# Autodesk Inventor assembly: Degree60CoffeeTable
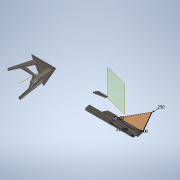
[picture p0: Inventor's stored thumbnail of the model, 180x180]
Saved by Autodesk Inventor 2022 (Build 260153000, 153)
## iProperties
Created: 2022-01-06
Part Number: Degree60CoffeeTable
Document SubType Name: Assembly
Designer: dangl
Author: dangl
## Documents named in this file (4)
- C:\Users\dangl\Documents\WoodWork\Degree60CoffeeTable\Degree60CoffeeTable.iam
- C:\Users\dangl\Documents\WoodWork\Degree60CoffeeTable\TableTop.ipt
- C:\Users\dangl\Documents\WoodWork\Degree60CoffeeTable\Leg.ipt
- C:\Users\dangl\Documents\WoodWork\Degree60CoffeeTable\LegConnector.ipt
## Components (17 placed, 3 different names)
1. TableTop:1 — Flush:1, Flush:2, Flush:3, Flush:5
2. Leg:6 — Mate:9, Mate:10, Flush:6, Flush:10, Mate:17
3. Leg:8 — Mate:6, Mate:10, Flush:6, Flush:8, Mate:12, Mate:16
4. LegConnector:6 — Mate:3, Mate:15, Mate:16
5. LegConnector:8 — Mate:5, Mate:15, Flush:13
6. Leg:9 — Flush:9, Flush:10, Mate:12
7. Leg:10 — Flush:8, Flush:9, Mate:14
8. Leg:11 — Mate:14
9. Leg:12 — Flush:13, Flush:14
10. LegConnector:9
11. TableTop:2 — Flush:14
12. Leg:1 — Flush:1
13. Leg:2
14. Leg:3
15. LegConnector:1 — Flush:4, Flush:5
16. LegConnector:2
17. LegConnector:3
## Component patterns: (3 elements, first: Leg:1), (3 elements, first: LegConnector:1)
## Relationships (29: Flush 14, Mate 14, Symmetry 1)
- Flush:1: TableTop:1 ↔ Leg:1
- Flush:2: TableTop:1
- Flush:3: TableTop:1
- Symmetry:1
- Mate:1
- Mate:2
- Flush:4: LegConnector:1
- Flush:5: TableTop:1 ↔ LegConnector:1
- Mate:3: LegConnector:6
- Mate:5: LegConnector:8
- Mate:6: Leg:8
- Mate:9: Leg:6
- Mate:10 (6.35 mm): Leg:6 ↔ Leg:8
- Flush:6: Leg:6 ↔ Leg:8
- [Mate] (6.35 mm): Leg:9 ↔ Leg:10
- [Flush]: Leg:9 ↔ Leg:10
- Flush:8: Leg:8 ↔ Leg:10
- Flush:9: Leg:9 ↔ Leg:10
- Flush:10: Leg:6 ↔ Leg:9
- Mate:12 (6.35 mm): Leg:8 ↔ Leg:9
- [Mate] (6.35 mm): Leg:11 ↔ Leg:12
- [Flush]: Leg:11 ↔ Leg:12
- [Flush]: Leg:11 ↔ Leg:12
- Mate:14 (6.35 mm): Leg:10 ↔ Leg:11
- Mate:15 (6.35 mm): LegConnector:6 ↔ LegConnector:8
- Mate:16 (6.35 mm): Leg:8 ↔ LegConnector:6
- Mate:17: Leg:6
- Flush:13: LegConnector:8 ↔ Leg:12
- Flush:14: Leg:12 ↔ TableTop:2
## Named parameters: d22_d20 = 6.35 mm, d23_d21 = 0 mm, d28_d22_d20 = 6.35 mm, d29_d23_d21 = 0 mm, d30_d25 = 0 mm
